# Autodesk Inventor assembly: robot_base
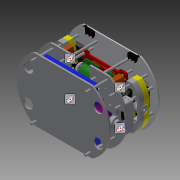
[picture p0: Inventor's stored thumbnail of the model, 180x180]
Saved by Autodesk Inventor 2015 (Build 190159000, 159)
## iProperties
Created: 2015-07-19
Part Number: robot_base
Document SubType Name: Assembly
Designer: astralien3000
Author: astralien3000
## Documents named in this file (15)
- C:\Users\astralien3000\Desktop\ceres\meca\v2016\robot_base.iam
- C:\Users\astralien3000\Desktop\ceres\meca\v2016\base.ipt
- C:\Users\astralien3000\Desktop\ceres\meca\v2016\odometer_block.iam
- C:\Users\astralien3000\Desktop\ceres\meca\v2016\wheel_block.iam
- C:\Users\astralien3000\Desktop\ceres\meca\lib\struct\vis_6mm_100mm.ipt
- C:\Users\astralien3000\Desktop\ceres\meca\lib\struct\patin_d18mm_e6mm.ipt
- C:\Users\astralien3000\Desktop\ceres\meca\v2016\motor.iam
- C:\Users\astralien3000\Desktop\ceres\meca\v2016\middle_base.ipt
- C:\Users\astralien3000\Desktop\ceres\meca\v2016\tendeur_block.iam
- C:\Users\astralien3000\Desktop\ceres\meca\lib\sensor\bumper.ipt
- C:\Users\astralien3000\Desktop\ceres\meca\lib\struct\vis_6mm_60mm.ipt
- C:\Users\astralien3000\Desktop\ceres\meca\v2016\top_base.ipt
- C:\Users\astralien3000\Desktop\ceres\meca\lib\battery\lipo2s.ipt
- C:\Users\astralien3000\Desktop\ceres\meca\v2016\gp2_block.iam
- C:\Users\astralien3000\Desktop\ceres\meca\v2016\rolling_base_board.ipt
## Components (45 placed, 14 different names)
1. base:1 — Placage:1, Affleurement:1, Placage:3, Placage:4, Placage:5, Placage:6, Placage:7, Placage:8, Placage:9, Placage:10, Placage:11, Placage:12, Placage:13, Placage:14, Placage:15, Placage:16, Placage:17, Placage:18, Placage:19, Placage:20, Placage:21, Placage:22, Placage:23, Placage:24, Placage:25, Placage:26, Placage:27, Placage:28, Placage:29, Placage:30, Placage:31, Placage:32, Placage:33, Placage:34, Placage:35, Placage:36, Placage:37, Placage:38, Placage:39, Placage:40, Placage:45, Placage:78, Placage:79, Placage:80, Placage:81, Placage:82, Placage:83, Placage:84, Placage:85, Placage:86, Placage:87, Placage:88, Placage:89, Placage:92, Placage:93, Placage:96, Placage:97, Placage:116
2. odometer_block:1 [sub-assembly] — Placage:3, Placage:4, Tangente:3
3. wheel_block:1 [sub-assembly] — Placage:5, Placage:6, Tangente:1
4. wheel_block:2 [sub-assembly] — Placage:7, Placage:8, Tangente:2
5. vis_6mm_100mm:1 — Placage:23, Placage:29, Placage:74
6. vis_6mm_100mm:2 — Placage:21, Placage:27
7. vis_6mm_100mm:3 — Placage:22, Placage:28, Placage:73
8. vis_6mm_100mm:4 — Placage:24, Placage:30
9. vis_6mm_100mm:5 — Placage:18, Placage:26
10. vis_6mm_100mm:6 — Placage:20, Placage:31, Placage:43
11. vis_6mm_100mm:7 — Placage:17, Placage:25, Placage:44
12. vis_6mm_100mm:8 — Placage:19, Placage:32
13. vis_6mm_100mm:9 — Placage:9, Placage:13
14. vis_6mm_100mm:10 — Placage:10, Placage:14, Placage:75
15. vis_6mm_100mm:11 — Placage:11, Placage:15, Placage:76
16. vis_6mm_100mm:12 — Placage:12, Placage:16
17. patin_d18mm_e6mm:1 — Placage:35, Placage:37
18. patin_d18mm_e6mm:2 — Placage:33, Placage:40, Tangente:2, Tangente:3
19. patin_d18mm_e6mm:3 — Placage:34, Placage:39, Tangente:1
20. patin_d18mm_e6mm:4 — Placage:36, Placage:38
21. motor:1 [sub-assembly] — Placage:49, Placage:50, Placage:51, Tangente:5, Tangente:6
22. motor:2 [sub-assembly] — Placage:46, Placage:47, Placage:48, Tangente:4
23. middle_base:1 — Placage:43, Placage:44, Placage:45, Placage:46, Placage:47, Placage:48, Placage:49, Placage:50, Placage:51, Placage:72, Placage:77, Placage:90, Placage:91, Placage:94, Placage:95, Placage:98, Placage:99, Placage:100, Placage:101, Placage:102, Placage:103, Placage:104, Placage:105, Placage:112, Placage:113, Placage:114, Placage:115, Placage:117, Placage:118, Placage:119, Placage:120, Placage:121, Placage:122, Placage:123, Placage:124, Placage:125
24. tendeur_block:1 [sub-assembly] — Placage:72, Placage:73, Placage:74
25. tendeur_block:2 [sub-assembly] — Placage:75, Placage:76, Placage:77
26. bumper:1 — Placage:78, Placage:79, Placage:80
27. bumper:2 — Placage:87, Placage:88, Placage:89
28. bumper:3 — Placage:81, Placage:82, Placage:83
29. bumper:4 — Placage:84, Placage:85, Placage:86
30. vis_6mm_100mm:13 — Placage:94, Placage:96
31. vis_6mm_100mm:14 — Placage:91, Placage:93
32. vis_6mm_100mm:15 — Placage:95, Placage:97
33. vis_6mm_100mm:16 — Placage:90, Placage:92
34. vis_6mm_60mm:1 — Placage:100, Placage:103, Placage:109
35. vis_6mm_60mm:2 — Placage:99, Placage:105, Placage:108
36. vis_6mm_60mm:3 — Placage:101, Placage:102, Placage:107
37. vis_6mm_60mm:4 — Placage:98, Placage:104, Placage:106
38. top_base:1 — Placage:106, Placage:107, Placage:108, Placage:109, Tangente:4, Placage:110, Placage:111
39. lipo2s:1 — Placage:110, Tangente:5
40. lipo2s:2 — Placage:111, Tangente:6
41. gp2_block:1 [sub-assembly] — Placage:117, Placage:118
42. gp2_block:2 [sub-assembly] — Placage:119, Placage:120
43. gp2_block:3 [sub-assembly] — Placage:114, Placage:115
44. gp2_block:4 [sub-assembly] — Placage:112, Placage:113
45. rolling_base_board:1 — Placage:121, Placage:122, Placage:123, Placage:124, Placage:125
## Relationships (109: Mate 102, Tangent 6, Flush 1)
- Placage:1 [Mate]: base:1
- Affleurement:1 [Flush]: base:1
- Placage:3 [Mate]: base:1 ↔ odometer_block:1
- Placage:4 [Mate]: base:1 ↔ odometer_block:1
- Placage:5 [Mate]: base:1 ↔ wheel_block:1
- Placage:6 [Mate]: base:1 ↔ wheel_block:1
- Placage:7 [Mate]: base:1 ↔ wheel_block:2
- Placage:8 [Mate]: base:1 ↔ wheel_block:2
- Placage:9 [Mate]: base:1 ↔ vis_6mm_100mm:9
- Placage:10 [Mate]: base:1 ↔ vis_6mm_100mm:10
- Placage:11 [Mate]: base:1 ↔ vis_6mm_100mm:11
- Placage:12 [Mate]: base:1 ↔ vis_6mm_100mm:12
- Placage:13 [Mate]: base:1 ↔ vis_6mm_100mm:9
- Placage:14 [Mate]: base:1 ↔ vis_6mm_100mm:10
- Placage:15 [Mate]: base:1 ↔ vis_6mm_100mm:11
- Placage:16 [Mate]: base:1 ↔ vis_6mm_100mm:12
- Placage:17 [Mate]: base:1 ↔ vis_6mm_100mm:7
- Placage:18 [Mate]: base:1 ↔ vis_6mm_100mm:5
- Placage:19 [Mate]: base:1 ↔ vis_6mm_100mm:8
- Placage:20 [Mate]: base:1 ↔ vis_6mm_100mm:6
- Placage:21 [Mate]: base:1 ↔ vis_6mm_100mm:2
- Placage:22 [Mate]: base:1 ↔ vis_6mm_100mm:3
- Placage:23 [Mate]: base:1 ↔ vis_6mm_100mm:1
- Placage:24 [Mate]: base:1 ↔ vis_6mm_100mm:4
- Placage:25 [Mate]: base:1 ↔ vis_6mm_100mm:7
- Placage:26 [Mate]: base:1 ↔ vis_6mm_100mm:5
- Placage:27 [Mate]: base:1 ↔ vis_6mm_100mm:2
- Placage:28 [Mate]: base:1 ↔ vis_6mm_100mm:3
- Placage:29 [Mate]: base:1 ↔ vis_6mm_100mm:1
- Placage:30 [Mate]: base:1 ↔ vis_6mm_100mm:4
- Placage:31 [Mate]: base:1 ↔ vis_6mm_100mm:6
- Placage:32 [Mate]: base:1 ↔ vis_6mm_100mm:8
- Placage:33 [Mate]: base:1 ↔ patin_d18mm_e6mm:2
- Placage:34 [Mate]: base:1 ↔ patin_d18mm_e6mm:3
- Placage:35 [Mate]: base:1 ↔ patin_d18mm_e6mm:1
- Placage:36 [Mate]: base:1 ↔ patin_d18mm_e6mm:4
- Placage:37 [Mate]: base:1 ↔ patin_d18mm_e6mm:1
- Placage:38 [Mate]: base:1 ↔ patin_d18mm_e6mm:4
- Placage:39 [Mate]: base:1 ↔ patin_d18mm_e6mm:3
- Placage:40 [Mate]: base:1 ↔ patin_d18mm_e6mm:2
- Tangente:1: wheel_block:1 ↔ patin_d18mm_e6mm:3
- Tangente:2: wheel_block:2 ↔ patin_d18mm_e6mm:2
- Tangente:3: odometer_block:1 ↔ patin_d18mm_e6mm:2
- Placage:43 [Mate]: vis_6mm_100mm:6 ↔ middle_base:1
- Placage:44 [Mate]: vis_6mm_100mm:7 ↔ middle_base:1
- Placage:45 [Mate] (80 mm): base:1 ↔ middle_base:1
- Placage:46 [Mate]: motor:2 ↔ middle_base:1
- Placage:47 [Mate]: motor:2 ↔ middle_base:1
- Placage:48 [Mate]: motor:2 ↔ middle_base:1
- Placage:49 [Mate]: motor:1 ↔ middle_base:1
- Placage:50 [Mate]: motor:1 ↔ middle_base:1
- Placage:51 [Mate]: motor:1 ↔ middle_base:1
- Placage:72 [Mate]: middle_base:1 ↔ tendeur_block:1
- Placage:73 [Mate]: vis_6mm_100mm:3 ↔ tendeur_block:1
- Placage:74 [Mate]: vis_6mm_100mm:1 ↔ tendeur_block:1
- Placage:75 [Mate]: vis_6mm_100mm:10 ↔ tendeur_block:2
- Placage:76 [Mate]: vis_6mm_100mm:11 ↔ tendeur_block:2
- Placage:77 [Mate]: middle_base:1 ↔ tendeur_block:2
- Placage:78 [Mate]: base:1 ↔ bumper:1
- Placage:79 [Mate]: base:1 ↔ bumper:1
- Placage:80 [Mate]: base:1 ↔ bumper:1
- Placage:81 [Mate]: base:1 ↔ bumper:3
- Placage:82 [Mate]: base:1 ↔ bumper:3
- Placage:83 [Mate]: base:1 ↔ bumper:3
- Placage:84 [Mate]: base:1 ↔ bumper:4
- Placage:85 [Mate]: base:1 ↔ bumper:4
- Placage:86 [Mate]: base:1 ↔ bumper:4
- Placage:87 [Mate]: base:1 ↔ bumper:2
- Placage:88 [Mate]: base:1 ↔ bumper:2
- Placage:89 [Mate]: base:1 ↔ bumper:2
- Placage:90 [Mate]: middle_base:1 ↔ vis_6mm_100mm:16
- Placage:91 [Mate]: middle_base:1 ↔ vis_6mm_100mm:14
- Placage:92 [Mate]: base:1 ↔ vis_6mm_100mm:16
- Placage:93 [Mate]: base:1 ↔ vis_6mm_100mm:14
- Placage:94 [Mate]: middle_base:1 ↔ vis_6mm_100mm:13
- Placage:95 [Mate]: middle_base:1 ↔ vis_6mm_100mm:15
- Placage:96 [Mate]: base:1 ↔ vis_6mm_100mm:13
- Placage:97 [Mate]: base:1 ↔ vis_6mm_100mm:15
- Placage:98 [Mate]: middle_base:1 ↔ vis_6mm_60mm:4
- Placage:99 [Mate]: middle_base:1 ↔ vis_6mm_60mm:2
- Placage:100 [Mate]: middle_base:1 ↔ vis_6mm_60mm:1
- Placage:101 [Mate]: middle_base:1 ↔ vis_6mm_60mm:3
- Placage:102 [Mate]: middle_base:1 ↔ vis_6mm_60mm:3
- Placage:103 [Mate]: middle_base:1 ↔ vis_6mm_60mm:1
- Placage:104 [Mate]: middle_base:1 ↔ vis_6mm_60mm:4
- Placage:105 [Mate]: middle_base:1 ↔ vis_6mm_60mm:2
- Placage:106 [Mate]: vis_6mm_60mm:4 ↔ top_base:1
- Placage:107 [Mate]: vis_6mm_60mm:3 ↔ top_base:1
- Placage:108 [Mate]: vis_6mm_60mm:2 ↔ top_base:1
- Placage:109 [Mate]: vis_6mm_60mm:1 ↔ top_base:1
- Tangente:4: motor:2 ↔ top_base:1
- Placage:110 [Mate]: top_base:1 ↔ lipo2s:1
- Tangente:5: motor:1 ↔ lipo2s:1
- Placage:111 [Mate]: top_base:1 ↔ lipo2s:2
- Tangente:6: motor:1 ↔ lipo2s:2
- Placage:112 [Mate]: middle_base:1 ↔ gp2_block:4
- Placage:113 [Mate]: middle_base:1 ↔ gp2_block:4
- Placage:114 [Mate]: middle_base:1 ↔ gp2_block:3
- Placage:115 [Mate]: middle_base:1 ↔ gp2_block:3
- Placage:116 [Mate]: base:1
- Placage:117 [Mate]: middle_base:1 ↔ gp2_block:1
- Placage:118 [Mate]: middle_base:1 ↔ gp2_block:1
- Placage:119 [Mate]: middle_base:1 ↔ gp2_block:2
- Placage:120 [Mate]: middle_base:1 ↔ gp2_block:2
- Placage:121 [Mate]: middle_base:1 ↔ rolling_base_board:1
- Placage:122 [Mate]: middle_base:1 ↔ rolling_base_board:1
- Placage:123 [Mate]: middle_base:1 ↔ rolling_base_board:1
- Placage:124 [Mate]: middle_base:1 ↔ rolling_base_board:1
- Placage:125 [Mate] (5 mm): middle_base:1 ↔ rolling_base_board:1
